# Autodesk Inventor assembly: 円盤
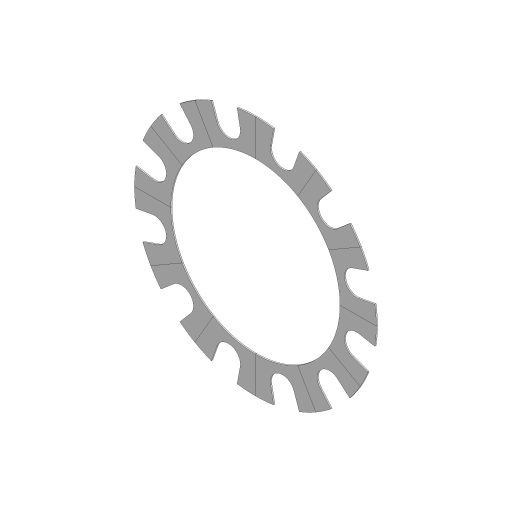
[picture p0: Inventor's stored thumbnail of the model, 512x512]
Saved by Autodesk Inventor 2023 (Build 270158000, 158)
## iProperties
Created: 2022-09-02
Part Number: 円盤
Document SubType Name: Assembly
Designer: monst
Author: monst
## Documents named in this file (2)
- D:\VENUSFOUNTAIN\Assets\円盤.iam
- D:\VENUSFOUNTAIN\Assets\円盤1.ipt
## Components (12 placed, 1 different names)
1. 円盤1:1 — メイト:1, メイト:2, フラッシュ:1, フラッシュ:2, メイト:3, メイト:4
2. 円盤1:2 — フラッシュ:2, メイト:3, メイト:4, フラッシュ:9, メイト:17, メイト:18
3. 円盤1:3 — メイト:1, メイト:2, フラッシュ:1
4. 円盤1:4 — フラッシュ:3, メイト:5, メイト:6
5. 円盤1:5 — フラッシュ:3, メイト:5, メイト:6, フラッシュ:4, メイト:7, メイト:8
6. 円盤1:6 — フラッシュ:4, メイト:7, メイト:8, フラッシュ:11, メイト:21, メイト:22
7. 円盤1:7 — フラッシュ:7, メイト:13, メイト:14, フラッシュ:9, メイト:17, メイト:18
8. 円盤1:8 — フラッシュ:7, フラッシュ:8, メイト:15, メイト:16, フラッシュ:10, メイト:19, メイト:20
9. 円盤1:9 — フラッシュ:8, メイト:13, メイト:14, メイト:15, メイト:16
10. 円盤1:10 — フラッシュ:6, メイト:11, メイト:12, フラッシュ:10, メイト:19, メイト:20
11. 円盤1:11 — フラッシュ:5, メイト:9, メイト:10, フラッシュ:6, メイト:11, メイト:12
12. 円盤1:12 — フラッシュ:5, メイト:9, メイト:10, フラッシュ:11, メイト:21, メイト:22
## Relationships (33: Mate 22, Flush 11)
- メイト:1 [Mate]: 円盤1:1 ↔ 円盤1:3
- メイト:2 [Mate]: 円盤1:1 ↔ 円盤1:3
- フラッシュ:1 [Flush]: 円盤1:1 ↔ 円盤1:3
- フラッシュ:2 [Flush]: 円盤1:1 ↔ 円盤1:2
- メイト:3 [Mate]: 円盤1:1 ↔ 円盤1:2
- メイト:4 [Mate]: 円盤1:1 ↔ 円盤1:2
- フラッシュ:3 [Flush]: 円盤1:4 ↔ 円盤1:5
- メイト:5 [Mate]: 円盤1:4 ↔ 円盤1:5
- メイト:6 [Mate]: 円盤1:4 ↔ 円盤1:5
- フラッシュ:4 [Flush]: 円盤1:5 ↔ 円盤1:6
- メイト:7 [Mate]: 円盤1:5 ↔ 円盤1:6
- メイト:8 [Mate]: 円盤1:5 ↔ 円盤1:6
- フラッシュ:5 [Flush]: 円盤1:11 ↔ 円盤1:12
- メイト:9 [Mate]: 円盤1:11 ↔ 円盤1:12
- メイト:10 [Mate]: 円盤1:11 ↔ 円盤1:12
- フラッシュ:6 [Flush]: 円盤1:10 ↔ 円盤1:11
- メイト:11 [Mate]: 円盤1:10 ↔ 円盤1:11
- メイト:12 [Mate]: 円盤1:10 ↔ 円盤1:11
- フラッシュ:7 [Flush]: 円盤1:7 ↔ 円盤1:8
- フラッシュ:8 [Flush]: 円盤1:8 ↔ 円盤1:9
- メイト:13 [Mate]: 円盤1:7 ↔ 円盤1:9
- メイト:14 [Mate]: 円盤1:7 ↔ 円盤1:9
- メイト:15 [Mate]: 円盤1:8 ↔ 円盤1:9
- メイト:16 [Mate]: 円盤1:8 ↔ 円盤1:9
- フラッシュ:9 [Flush]: 円盤1:2 ↔ 円盤1:7
- メイト:17 [Mate]: 円盤1:2 ↔ 円盤1:7
- メイト:18 [Mate]: 円盤1:2 ↔ 円盤1:7
- フラッシュ:10 [Flush]: 円盤1:8 ↔ 円盤1:10
- メイト:19 [Mate]: 円盤1:8 ↔ 円盤1:10
- メイト:20 [Mate]: 円盤1:8 ↔ 円盤1:10
- フラッシュ:11 [Flush]: 円盤1:6 ↔ 円盤1:12
- メイト:21 [Mate]: 円盤1:6 ↔ 円盤1:12
- メイト:22 [Mate]: 円盤1:6 ↔ 円盤1:12
